# Autodesk Inventor assembly: Mini V Gantry Kit
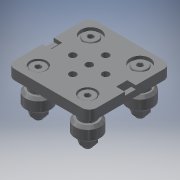
[picture p0: Inventor's stored thumbnail of the model, 180x180]
Saved by Autodesk Inventor 2019 (Build 230136000, 136)
## iProperties
Created: 2019-09-26
Part Number: Mini V Gantry Kit
Document SubType Name: Assembly
Designer: zhanb
Sending System: Autodesk Translation Framework v8.6.0.1094
Preprocessor: ST-DEVELOPER v18
Title: /Users/ayahni/Downloads/Mini V Gantry Kit.step
## Documents named in this file (9)
- F:\3D Objects\Inventor\Coursework\ECE HyperRail\Gantry\Mini V Gantry Kit.iam
- F:\3D Objects\Inventor\Coursework\ECE HyperRail\Gantry\Low Profile Screw M5 v1.ipt
- F:\3D Objects\Inventor\Coursework\ECE HyperRail\Gantry\Nylon Insert Lock Nut M5 v1.ipt
- F:\3D Objects\Inventor\Coursework\ECE HyperRail\Gantry\Precision Shim 8 x 5 x 1 v1.ipt
- F:\3D Objects\Inventor\Coursework\ECE HyperRail\Gantry\Eccentric Spacer 6mm v1.ipt
- F:\3D Objects\Inventor\Coursework\ECE HyperRail\Gantry\Aluminum Spacer 6mm v1.ipt
- F:\3D Objects\Inventor\Coursework\ECE HyperRail\Gantry\Mini V Wheel Plate v1.ipt
- F:\3D Objects\Inventor\Coursework\ECE HyperRail\Gantry\Delrin Mini V Wheel v1.ipt
- F:\3D Objects\Inventor\Coursework\ECE HyperRail\Gantry\Ball Bearing 5 x 10 x 4.2 v1.ipt
## Components (29 placed, 8 different names)
1. Aluminum Spacer 6mm v1:2
2. Mini V Wheel Plate v1:1 — Mate:5, Mate:9, Mate:10, Mate:23
3. Ball Bearing 5 x 10 x 4.2 v1:3 — Mate:1, Flush:2
4. Ball Bearing 5 x 10 x 4.2 v1:4 — Mate:1, Flush:1, Mate:2, Mate:3, Mate:11
5. Delrin Mini V Wheel v1:2 — Flush:1, Flush:2, Mate:2, Mate:4, Mate:7, Mate:8, Mate:9
6. Low Profile Screw M5 v1:5 — Mate:6, Mate:7, Mate:10, Mate:12, Flush:5
7. Nylon Insert Lock Nut M5 v1:6 — Mate:3, Mate:4
8. Precision Shim 8 x 5 x 1 v1:5 — Mate:11, Mate:12
9. Eccentric Spacer 6mm v1:3 — Mate:5, Mate:6, Mate:8
10. Precision Shim 8 x 5 x 1 v1:6
11. Nylon Insert Lock Nut M5 v1:7
12. Low Profile Screw M5 v1:6
13. Delrin Mini V Wheel v1:3
14. Ball Bearing 5 x 10 x 4.2 v1:5
15. Ball Bearing 5 x 10 x 4.2 v1:6
16. Ball Bearing 5 x 10 x 4.2 v1:7
17. Ball Bearing 5 x 10 x 4.2 v1:8
18. Delrin Mini V Wheel v1:4
19. Precision Shim 8 x 5 x 1 v1:7
20. Nylon Insert Lock Nut M5 v1:8
21. Low Profile Screw M5 v1:7
22. Aluminum Spacer 6mm v1:3
23. Ball Bearing 5 x 10 x 4.2 v1:9 — Mate:18, Mate:19, Mate:21
24. Ball Bearing 5 x 10 x 4.2 v1:10 — Mate:20, Flush:4, Mate:22
25. Low Profile Screw M5 v1:8 — Mate:18, Flush:3, Flush:5
26. Nylon Insert Lock Nut M5 v1:9 — Mate:20, Flush:3
27. Precision Shim 8 x 5 x 1 v1:8 — Mate:19
28. Eccentric Spacer 6mm v1:4 — Mate:21
29. Delrin Mini V Wheel v1:5 — Flush:4, Mate:22, Mate:23
## Relationships (28: Mate 23, Flush 5)
- Mate:1: Ball Bearing 5 x 10 x 4.2 v1:3 ↔ Ball Bearing 5 x 10 x 4.2 v1:4
- Flush:1: Ball Bearing 5 x 10 x 4.2 v1:4 ↔ Delrin Mini V Wheel v1:2
- Flush:2: Ball Bearing 5 x 10 x 4.2 v1:3 ↔ Delrin Mini V Wheel v1:2
- Mate:2: Ball Bearing 5 x 10 x 4.2 v1:4 ↔ Delrin Mini V Wheel v1:2
- Mate:3: Ball Bearing 5 x 10 x 4.2 v1:4 ↔ Nylon Insert Lock Nut M5 v1:6
- Mate:4: Delrin Mini V Wheel v1:2 ↔ Nylon Insert Lock Nut M5 v1:6
- Mate:5: Mini V Wheel Plate v1:1 ↔ Eccentric Spacer 6mm v1:3
- Mate:6: Low Profile Screw M5 v1:5 ↔ Eccentric Spacer 6mm v1:3
- Mate:7: Delrin Mini V Wheel v1:2 ↔ Low Profile Screw M5 v1:5
- Mate:8: Delrin Mini V Wheel v1:2 ↔ Eccentric Spacer 6mm v1:3
- Mate:9: Mini V Wheel Plate v1:1 ↔ Delrin Mini V Wheel v1:2
- Mate:10: Mini V Wheel Plate v1:1 ↔ Low Profile Screw M5 v1:5
- Mate:11: Ball Bearing 5 x 10 x 4.2 v1:4 ↔ Precision Shim 8 x 5 x 1 v1:5
- Mate:12: Low Profile Screw M5 v1:5 ↔ Precision Shim 8 x 5 x 1 v1:5
- [Mate]: Ball Bearing 5 x 10 x 4.2 v1:9 ↔ Ball Bearing 5 x 10 x 4.2 v1:10
- [Mate]: Ball Bearing 5 x 10 x 4.2 v1:10 ↔ Nylon Insert Lock Nut M5 v1:9
- [Mate]: Low Profile Screw M5 v1:8 ↔ Eccentric Spacer 6mm v1:4
- [Mate]: Ball Bearing 5 x 10 x 4.2 v1:10 ↔ Precision Shim 8 x 5 x 1 v1:8
- [Mate]: Low Profile Screw M5 v1:8 ↔ Precision Shim 8 x 5 x 1 v1:8
- Mate:18: Ball Bearing 5 x 10 x 4.2 v1:9 ↔ Low Profile Screw M5 v1:8
- Mate:19: Ball Bearing 5 x 10 x 4.2 v1:9 ↔ Precision Shim 8 x 5 x 1 v1:8
- Mate:20: Ball Bearing 5 x 10 x 4.2 v1:10 ↔ Nylon Insert Lock Nut M5 v1:9
- Mate:21: Ball Bearing 5 x 10 x 4.2 v1:9 ↔ Eccentric Spacer 6mm v1:4
- Flush:3 (-1.7 mm): Low Profile Screw M5 v1:8 ↔ Nylon Insert Lock Nut M5 v1:9
- Flush:4: Ball Bearing 5 x 10 x 4.2 v1:10 ↔ Delrin Mini V Wheel v1:5
- Mate:22: Ball Bearing 5 x 10 x 4.2 v1:10 ↔ Delrin Mini V Wheel v1:5
- Mate:23: Mini V Wheel Plate v1:1 ↔ Delrin Mini V Wheel v1:5
- Flush:5: Low Profile Screw M5 v1:5 ↔ Low Profile Screw M5 v1:8
## Named parameters: d14_d13 = 0 mm, d15_d0 = 0 mm, d16_d4 = 0 mm, d17_d7 = 0 mm, d18_d12 = 0 mm
